# Autodesk Inventor assembly: Wide_2017_chassis
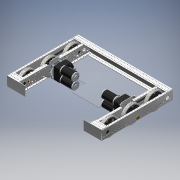
[picture p0: Inventor's stored thumbnail of the model, 180x180]
Saved by Autodesk Inventor 2017 (Build 210142000, 142)
## iProperties
Created: 2017-01-13
Part Number: Wide_2017_chassis
Description: STEP AP203
Document SubType Name: Assembly
Designer: Ben
Sending System: SolidWorks 2015
Preprocessor: SwSTEP 2.0
Title: AM14U_wide_2017_chassis.STEP
Revision Number: ANY
## Documents named in this file (6)
- C:\Users\Ben\Desktop\Projects\2017 Robot\Frame\Wide_2017_chassis.iam
- C:\Users\Ben\Desktop\Projects\2017 Robot\Frame\AM14U3 Wide Half.iam
- C:\Users\Ben\Desktop\Projects\2017 Robot\Frame\AM14U3 End Sheet Rev1.ipt
- C:\Users\Ben\Desktop\Projects\2017 Robot\Frame\AM14U3 Bumper End Sheet Short.ipt
- C:\Users\Ben\Desktop\Projects\2017 Robot\Frame\Vex Pro 3 Stage.iam
- C:\Users\Ben\Desktop\Projects\2017 Robot\Frame\Electronics Plate.ipt
## Components (8 placed, 7 different names)
1. AM14U3 Wide Half_1 [sub-assembly] — Mate:1, Mate:2, Angle:2, Flush:2, Insert:3, Insert:4, Symmetry:1, Insert:7, Insert:8
2. AM14U3 Wide Half_2 [sub-assembly] — Mate:3, Mate:4, Angle:1, Insert:1, Insert:2, Symmetry:1, Insert:5, Insert:6
3. AM14U3 End Sheet Rev1_3 — Flush:1, Mate:5, Insert:5, Insert:6, Insert:7, Insert:8, Mate:6
4. AM14U3 Bumper End Sheet Short_4 — Insert:3, Insert:4
5. AM14U3 Bumper End Sheet Short_5 — Insert:1, Insert:2, Flush:3
6. Vex Pro 3 Stage:1 [sub-assembly] — Mate:1, Mate:2, Angle:2
7. Vex Pro 3 Stage:2 [sub-assembly] — Mate:3, Mate:4, Angle:1
8. Electronics Plate:1 — Flush:1, Flush:2, Mate:5
## Relationships (20: Insert 8, Mate 6, Flush 3, Angle 2, Symmetry 1)
- Mate:1: AM14U3 Wide Half_1 ↔ Vex Pro 3 Stage:1
- Mate:2: AM14U3 Wide Half_1 ↔ Vex Pro 3 Stage:1
- Mate:3: AM14U3 Wide Half_2 ↔ Vex Pro 3 Stage:2
- Mate:4: AM14U3 Wide Half_2 ↔ Vex Pro 3 Stage:2
- Angle:1 (90 deg): AM14U3 Wide Half_2 ↔ Vex Pro 3 Stage:2
- Angle:2 (-90 deg): AM14U3 Wide Half_1 ↔ Vex Pro 3 Stage:1
- Flush:1: AM14U3 End Sheet Rev1_3 ↔ Electronics Plate:1
- Flush:2: AM14U3 Wide Half_1 ↔ Electronics Plate:1
- Mate:5 (25.4 mm): AM14U3 End Sheet Rev1_3 ↔ Electronics Plate:1
- Insert:1: AM14U3 Wide Half_2 ↔ AM14U3 Bumper End Sheet Short_5
- Insert:2: AM14U3 Wide Half_2 ↔ AM14U3 Bumper End Sheet Short_5
- Insert:3: AM14U3 Wide Half_1 ↔ AM14U3 Bumper End Sheet Short_4
- Insert:4: AM14U3 Wide Half_1 ↔ AM14U3 Bumper End Sheet Short_4
- Symmetry:1: AM14U3 Wide Half_1 ↔ AM14U3 Wide Half_2
- Insert:5: AM14U3 Wide Half_2 ↔ AM14U3 End Sheet Rev1_3
- Insert:6: AM14U3 Wide Half_2 ↔ AM14U3 End Sheet Rev1_3
- Insert:7: AM14U3 Wide Half_1 ↔ AM14U3 End Sheet Rev1_3
- Insert:8: AM14U3 Wide Half_1 ↔ AM14U3 End Sheet Rev1_3
- Mate:6 (50.8 mm): AM14U3 End Sheet Rev1_3
- Flush:3: AM14U3 Bumper End Sheet Short_5
